# Autodesk Inventor assembly: Print setup 11 inch
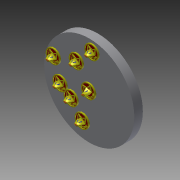
[picture p0: Inventor's stored thumbnail of the model, 180x180]
Saved by Autodesk Inventor 2014 (Build 180170000, 170)
## iProperties
Created: 2015-01-24
Part Number: Print setup 11 inch
Document SubType Name: Assembly
Designer: Spooner
Author: Spooner
## Documents named in this file (3)
- C:\Users\Spooner\Documents\Inventor\RoboCat\Print setup 11 inch.iam
- C:\Users\Spooner\Documents\Inventor\RoboCat\11 inch bed.ipt
- C:\Users\Spooner\Documents\Inventor\RoboCat\Full Pin.iam
## Components (8 placed, 2 different names)
1. 11 inch bed:1 — Insert:1, Mate:1, Mate:3, Mate:4, Mate:5, Mate:6, Mate:7
2. Full Pin:1 [sub-assembly] — Mate:1
3. Full Pin:2 [sub-assembly] — Mate:3
4. Full Pin:3 [sub-assembly] — Mate:4
5. Full Pin:4 [sub-assembly] — Mate:5
6. Full Pin:5 [sub-assembly] — Mate:6
7. Full Pin:6 [sub-assembly] — Mate:7
8. Full Pin:7 [sub-assembly] — Insert:1, Angle:1
## Relationships (8: Mate 6, Insert 1, Angle 1)
- Insert:1: 11 inch bed:1 ↔ Full Pin:7
- Angle:1 (180 deg): Full Pin:7
- Mate:1: 11 inch bed:1 ↔ Full Pin:1
- Mate:3: 11 inch bed:1 ↔ Full Pin:2
- Mate:4: 11 inch bed:1 ↔ Full Pin:3
- Mate:5: 11 inch bed:1 ↔ Full Pin:4
- Mate:6: 11 inch bed:1 ↔ Full Pin:5
- Mate:7: 11 inch bed:1 ↔ Full Pin:6
